# Autodesk Inventor assembly: 2905-0006-0008 assembly
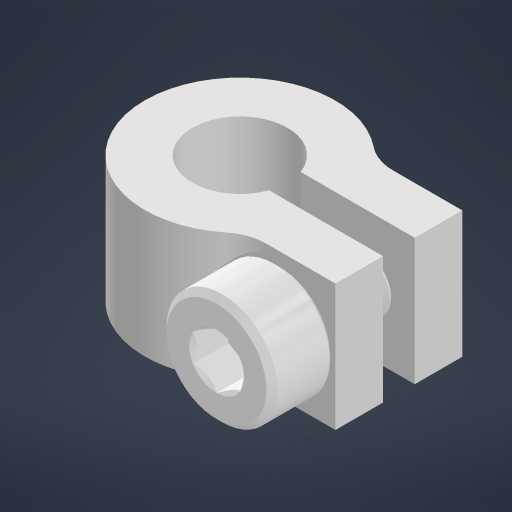
[picture p0: Inventor's stored thumbnail of the model, 512x512]
Saved by Autodesk Inventor 2023 (Build 270158000, 158)
## iProperties
Created: 2018-08-08
Part Number: 2905-0006-0008 assembly
Description: STEP AP203
Document SubType Name: Assembly
Designer: Arash
Sending System: SolidWorks 2016
Preprocessor: SwSTEP 2.0
Title: 2905-0006-0008 assembly.STEP
Revision Number: ANY
## Documents named in this file (3)
- C:\$WorkingFolder\Engineering Data\FTC_Parts_Library\goBilda\Motion\Collars\(6mm Bore, 8mm Length) 2905 Series Aluminum Clamping Collar.iam
- C:\$WorkingFolder\Engineering Data\FTC_Parts_Library\goBilda\Motion\Collars\Without Screw\2905-0006-0008.ipt
- C:\$WorkingFolder\Engineering Data\FTC_Parts_Library\ISO Standard Hardware\Screws\Sockethead Screws\Cap Screws\M4 x 0.7mm\(M4 x 0.7 x 8) Sockethead Cap Screw.ipt
## Components (2 placed, 2 different names)
1. 2905-0006-0008_1 — Mate:1, Mate:2
2. (M4 x 0.7 x 8) Sockethead Cap Screw:1 — Mate:1, Mate:2
## Relationships (2: Mate 2)
- Mate:1: 2905-0006-0008_1 ↔ (M4 x 0.7 x 8) Sockethead Cap Screw:1
- Mate:2: 2905-0006-0008_1 ↔ (M4 x 0.7 x 8) Sockethead Cap Screw:1
